# Autodesk Inventor assembly: Link2
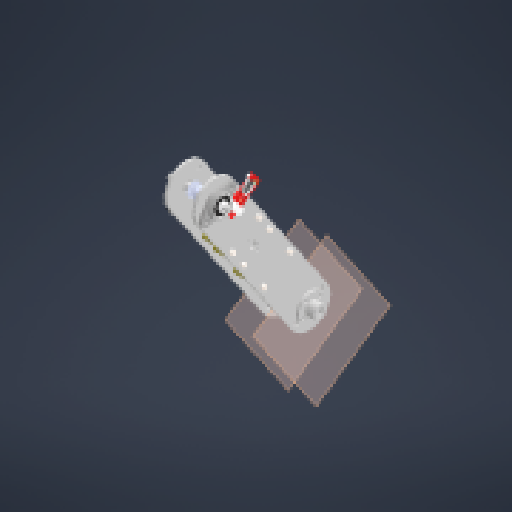
[picture p0: Inventor's stored thumbnail of the model, 512x512]
Saved by Autodesk Inventor 2023 (Build 270158000, 158)
## iProperties
Created: 2023-09-09
Part Number: Link2
Document SubType Name: Assembly
Designer: philo
Author: philo
## Documents named in this file (13)
- C:\Users\philo\OneDrive\Desktop\HK1-2024\TT ROBOT\02_3D_design_new\Link2.iam
- C:\Users\philo\OneDrive\Desktop\HK1-2024\TT ROBOT\02_3D_design_new\Link2Base.ipt
- C:\Users\philo\OneDrive\Desktop\HK1-2024\TT ROBOT\02_3D_design_new\goidoObi.ipt
- C:\Users\philo\OneDrive\Desktop\HK1-2024\TT ROBOT\02_3D_design_new\truc8mm.ipt
- C:\Users\philo\OneDrive\Desktop\HK1-2024\TT ROBOT\02_3D_design_new\GT2 Pulley 20 Tooth (ID6mm).ipt
- C:\Users\philo\OneDrive\Desktop\HK1-2024\TT ROBOT\02_3D_design_new\trudong3mm.ipt
- C:\Users\philo\OneDrive\Desktop\HK1-2024\TT ROBOT\02_3D_design_new\M3 x 5mm.ipt
- C:\Users\philo\OneDrive\Desktop\HK1-2024\TT ROBOT\02_3D_design_new\codinhtruc.ipt
- C:\Users\philo\OneDrive\Desktop\HK1-2024\TT ROBOT\02_3D_design_new\Dongco.iam
- C:\Users\philo\OneDrive\Desktop\HK1-2024\TT ROBOT\02_3D_design_new\limitswitch.ipt
- C:\Users\philo\OneDrive\Desktop\HK1-2024\TT ROBOT\02_3D_design_new\bulong5mmdai50.ipt
- C:\Users\philo\OneDrive\Desktop\HK1-2024\TT ROBOT\02_3D_design_new\oc5mm.ipt
- C:\Users\philo\OneDrive\Desktop\HK1-2024\TT ROBOT\02_3D_design_new\gt2smooth.ipt
## Components (38 placed, 12 different names)
1. oc5mm:1 — Mate:90, Mate:91
2. gt2smooth:1 — Mate:92, Mate:93
3. oc5mm:2 — Mate:94, Mate:95
4. oc5mm:3 — Mate:96, Mate:97
5. trudong3mm:1 — Mate:98, Mate:99
6. trudong3mm:2 — Mate:100, Mate:106, Mate:124
7. trudong3mm:3 — Mate:101, Mate:107
8. trudong3mm:7 — Mate:103, Mate:105, Mate:121
9. trudong3mm:8 — Mate:102, Mate:104
10. trudong3mm:9 — Mate:108, Mate:109, Mate:120
11. trudong3mm:10 — Mate:110, Mate:111
12. M3 x 5mm:1 — Mate:112, Mate:120
13. M3 x 5mm:2 — Mate:113, Mate:124
14. M3 x 5mm:4 — Mate:115, Mate:121
15. M3 x 5mm:5 — Mate:116, Mate:122
16. M3 x 5mm:6 — Mate:117, Mate:123
17. M3 x 5mm:7 — Mate:118, Mate:119
18. M3 x 5mm:8 — Mate:125, Mate:126
19. M3 x 5mm:9 — Mate:127, Mate:128
20. M3 x 5mm:11 — Mate:135, Mate:142
21. M3 x 5mm:12 — Mate:134, Mate:141
22. M3 x 5mm:13 — Mate:133, Mate:140
23. M3 x 5mm:14 — Mate:132, Mate:139
24. M3 x 5mm:15 — Mate:131, Mate:138
25. M3 x 5mm:16 — Mate:130, Mate:137
26. M3 x 5mm:17 — Mate:129, Mate:136
27. limitswitch:1 — Mate:86, Flush:5, Mate:87, Mate:125, Mate:127, Mate:128
28. GT2 Pulley 20 Tooth (ID6mm):2 — Mate:84, Mate:85
29. GT2 Pulley 20 Tooth (ID6mm):1 — Mate:80, Mate:81
30. Dongco:1 [sub-assembly] — Mate:78, Angle:3, Mate:79, Mate:80
31. Link2Base:2 — Mate:71, Mate:72, Mate:73, Mate:74, Mate:75, Angle:2, Mate:78, Mate:79, Mate:81, Mate:88, Flush:6, Mate:89, Mate:90, Mate:93, Mate:98, Mate:99, Mate:100, Mate:101, Mate:102, Mate:103, Mate:104, Mate:105, Mate:106, Mate:107, Mate:108, Mate:109, Mate:110, Mate:111, Mate:126, Mate:129, Mate:130, Mate:131, Mate:132, Mate:133, Mate:134, Mate:135, Mate:136, Mate:137, Mate:138, Mate:139, Mate:140, Mate:141, Mate:142
32. Link2Base:3 — Mate:68, Mate:69, Mate:70, Angle:3, Mate:82, Mate:83, Mate:85, Mate:86, Flush:5, Mate:94, Mate:96, Mate:112, Mate:113, Mate:115, Mate:116, Mate:117, Mate:118, Mate:119, Mate:122, Mate:123
33. goidoObi:2
34. truc8mm:1 — Mate:84, Mate:87
35. goidoObi:3 — Mate:74, Mate:75, Angle:2, Mate:82
36. codinhtruc:1 — Mate:68, Mate:69, Mate:70
37. codinhtruc:2 — Mate:71, Mate:72, Mate:73, Mate:83
38. bulong5mmdai50:1 — Mate:88, Flush:6, Mate:89, Mate:91, Mate:92, Mate:95, Mate:97
## Relationships (82: Mate 76, Angle 3, Flush 3)
- [Mate] (30 mm): Link2Base:2 ↔ Link2Base:3
- [Mate]: Link2Base:3 ↔ goidoObi:2
- [Mate]: Link2Base:3 ↔ goidoObi:2
- [Angle] (90 deg): Link2Base:3 ↔ goidoObi:2
- [Flush] (-5 mm): goidoObi:2 ↔ truc8mm:1
- [Mate]: goidoObi:2 ↔ truc8mm:1
- Mate:68: Link2Base:3 ↔ codinhtruc:1
- Mate:69: Link2Base:3 ↔ codinhtruc:1
- Mate:70: Link2Base:3 ↔ codinhtruc:1
- Mate:71: Link2Base:2 ↔ codinhtruc:2
- Mate:72: Link2Base:2 ↔ codinhtruc:2
- Mate:73: Link2Base:2 ↔ codinhtruc:2
- Mate:74: Link2Base:2 ↔ goidoObi:3
- Mate:75: Link2Base:2 ↔ goidoObi:3
- Angle:2 (0 deg): Link2Base:2 ↔ goidoObi:3
- Mate:78: Dongco:1 ↔ Link2Base:2
- Angle:3 (0 deg): Dongco:1 ↔ Link2Base:3
- Mate:79: Dongco:1 ↔ Link2Base:2
- Mate:80: GT2 Pulley 20 Tooth (ID6mm):1 ↔ Dongco:1
- Mate:81 (2 mm): GT2 Pulley 20 Tooth (ID6mm):1 ↔ Link2Base:2
- Mate:82: Link2Base:3 ↔ goidoObi:3
- Mate:83: Link2Base:3 ↔ codinhtruc:2
- Mate:84: GT2 Pulley 20 Tooth (ID6mm):2 ↔ truc8mm:1
- Mate:85 (7 mm): GT2 Pulley 20 Tooth (ID6mm):2 ↔ Link2Base:3
- Mate:86: limitswitch:1 ↔ Link2Base:3
- Flush:5 (25 mm): limitswitch:1 ↔ Link2Base:3
- Mate:87 (15 mm): limitswitch:1 ↔ truc8mm:1
- Mate:88 (2.5 mm): Link2Base:2 ↔ bulong5mmdai50:1
- Flush:6 (15 mm): Link2Base:2 ↔ bulong5mmdai50:1
- Mate:89: Link2Base:2 ↔ bulong5mmdai50:1
- Mate:90: oc5mm:1 ↔ Link2Base:2
- Mate:91: oc5mm:1 ↔ bulong5mmdai50:1
- Mate:92: gt2smooth:1 ↔ bulong5mmdai50:1
- Mate:93 (8 mm): gt2smooth:1 ↔ Link2Base:2
- Mate:94: oc5mm:2 ↔ Link2Base:3
- Mate:95: oc5mm:2 ↔ bulong5mmdai50:1
- Mate:96: oc5mm:3 ↔ Link2Base:3
- Mate:97: oc5mm:3 ↔ bulong5mmdai50:1
- Mate:98: trudong3mm:1 ↔ Link2Base:2
- Mate:99: trudong3mm:1 ↔ Link2Base:2
- Mate:100: trudong3mm:2 ↔ Link2Base:2
- Mate:101: trudong3mm:3 ↔ Link2Base:2
- Mate:102: trudong3mm:8 ↔ Link2Base:2
- Mate:103: trudong3mm:7 ↔ Link2Base:2
- Mate:104: trudong3mm:8 ↔ Link2Base:2
- Mate:105: trudong3mm:7 ↔ Link2Base:2
- Mate:106: trudong3mm:2 ↔ Link2Base:2
- Mate:107: trudong3mm:3 ↔ Link2Base:2
- Mate:108: trudong3mm:9 ↔ Link2Base:2
- Mate:109: trudong3mm:9 ↔ Link2Base:2
- Mate:110: trudong3mm:10 ↔ Link2Base:2
- Mate:111: trudong3mm:10 ↔ Link2Base:2
- Mate:112: M3 x 5mm:1 ↔ Link2Base:3
- Mate:113: M3 x 5mm:2 ↔ Link2Base:3
- Mate:115: M3 x 5mm:4 ↔ Link2Base:3
- Mate:116: M3 x 5mm:5 ↔ Link2Base:3
- Mate:117: M3 x 5mm:6 ↔ Link2Base:3
- Mate:118: M3 x 5mm:7 ↔ Link2Base:3
- Mate:119: M3 x 5mm:7 ↔ Link2Base:3
- Mate:120: trudong3mm:9 ↔ M3 x 5mm:1
- Mate:121: trudong3mm:7 ↔ M3 x 5mm:4
- Mate:122: M3 x 5mm:5 ↔ Link2Base:3
- Mate:123: M3 x 5mm:6 ↔ Link2Base:3
- Mate:124: trudong3mm:2 ↔ M3 x 5mm:2
- Mate:125: M3 x 5mm:8 ↔ limitswitch:1
- Mate:126: M3 x 5mm:8 ↔ Link2Base:2
- Mate:127: M3 x 5mm:9 ↔ limitswitch:1
- Mate:128: M3 x 5mm:9 ↔ limitswitch:1
- Mate:129: M3 x 5mm:17 ↔ Link2Base:2
- Mate:130: M3 x 5mm:16 ↔ Link2Base:2
- Mate:131: M3 x 5mm:15 ↔ Link2Base:2
- Mate:132: M3 x 5mm:14 ↔ Link2Base:2
- Mate:133: M3 x 5mm:13 ↔ Link2Base:2
- Mate:134: M3 x 5mm:12 ↔ Link2Base:2
- Mate:135: M3 x 5mm:11 ↔ Link2Base:2
- Mate:136: M3 x 5mm:17 ↔ Link2Base:2
- Mate:137: M3 x 5mm:16 ↔ Link2Base:2
- Mate:138: M3 x 5mm:15 ↔ Link2Base:2
- Mate:139: M3 x 5mm:14 ↔ Link2Base:2
- Mate:140: M3 x 5mm:13 ↔ Link2Base:2
- Mate:141: M3 x 5mm:12 ↔ Link2Base:2
- Mate:142: M3 x 5mm:11 ↔ Link2Base:2
